# Autodesk Inventor assembly: TrayFeeder
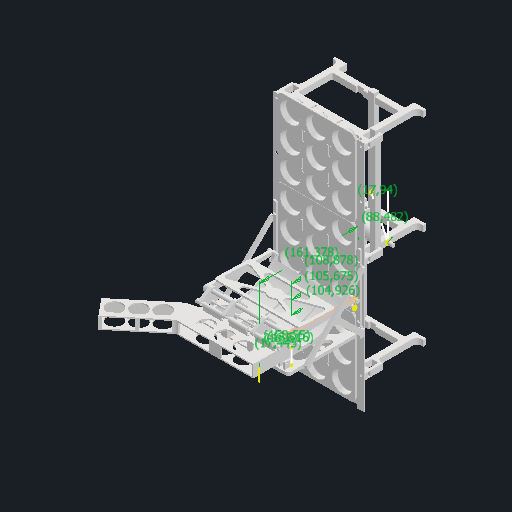
[picture p0: Inventor's stored thumbnail of the model, 512x512]
Saved by Autodesk Inventor 2026 (Build 300175050, 175E)
## iProperties
Created: 2026-05-01
Part Number: TrayFeeder
Document SubType Name: Assembly
Designer: frede
Author: frede
## Documents named in this file (18)
- C:\Users\sniel\OneDrive\SDU\4_Semester\Applied automation\AppliedAutomationProject\feeder\trayFeeder\TrayFeeder.iam
- C:\Users\sniel\OneDrive\SDU\4_Semester\Applied automation\AppliedAutomationProject\feeder\trayFeeder\TrayRail.ipt
- C:\Users\sniel\OneDrive\SDU\4_Semester\Applied automation\AppliedAutomationProject\feeder\trayFeeder\Tray.ipt
- C:\Users\sniel\OneDrive\SDU\4_Semester\Applied automation\AppliedAutomationProject\feeder\trayFeeder\TrayMainLegs.ipt
- C:\Users\sniel\OneDrive\SDU\4_Semester\Applied automation\AppliedAutomationProject\feeder\trayFeeder\Train.ipt
- C:\Users\sniel\OneDrive\SDU\4_Semester\Applied automation\AppliedAutomationProject\feeder\trayFeeder\TrainPullert.ipt
- C:\Users\sniel\OneDrive\SDU\4_Semester\Applied automation\AppliedAutomationProject\feeder\trayFeeder\TrainRail.ipt
- C:\Users\sniel\OneDrive\SDU\4_Semester\Applied automation\AppliedAutomationProject\feeder\trayFeeder\Spacer.ipt
- C:\Users\sniel\OneDrive\SDU\4_Semester\Applied automation\AppliedAutomationProject\feeder\trayFeeder\TrayMainLegs_toPistonWheel.ipt
- C:\Users\sniel\OneDrive\SDU\4_Semester\Applied automation\AppliedAutomationProject\feeder\trayFeeder\Crankshaft.ipt
- C:\Users\sniel\OneDrive\SDU\4_Semester\Applied automation\AppliedAutomationProject\feeder\trayFeeder\ParrallelShaft.ipt
- C:\Users\sniel\OneDrive\SDU\4_Semester\Applied automation\AppliedAutomationProject\feeder\trayFeeder\parrallelShaftPin.ipt
- C:\Users\sniel\OneDrive\SDU\4_Semester\Applied automation\AppliedAutomationProject\feeder\trayFeeder\gaffel.ipt
- C:\Users\sniel\OneDrive\SDU\4_Semester\Applied automation\AppliedAutomationProject\feeder\trayFeeder\ForkTop.ipt
- C:\Users\sniel\OneDrive\SDU\4_Semester\Applied automation\AppliedAutomationProject\feeder\trayFeeder\Ø6x40Shaft.ipt
- C:\Users\sniel\OneDrive\SDU\4_Semester\Applied automation\AppliedAutomationProject\feeder\trayFeeder\LegsStabilizer.ipt
- C:\Users\sniel\OneDrive\SDU\4_Semester\Applied automation\AppliedAutomationProject\feeder\trayFeeder\CoinFeeder.iam
- C:\Users\sniel\OneDrive\SDU\4_Semester\Applied automation\AppliedAutomationProject\feeder\trayFeeder\CoinFeederFoot.ipt
## Components (48 placed, 17 different names)
1. TrayRail:1 — Mate:1, Mate:2, Mate:3, Mate:6, Mate:7, Mate:8, Mate:12, Mate:13, Mate:17, Mate:18, Mate:22, Mate:83, Mate:84, Mate:85, Flush:3, Mate:150, Flush:4
2. Tray:1 — Mate:2, Mate:4, Mate:5, Flush:1, Flush:2
3. Tray:2 — Mate:3, Mate:4, Flush:2
4. Tray:3 — Mate:1, Mate:5, Mate:6, Mate:7, Flush:1
5. TrayMainLegs:1 — Mate:8, Mate:17, Mate:18, Mate:27, Mate:28, Mate:130, Mate:133, Mate:134
6. TrayMainLegs:5 — Mate:12, Mate:13, Mate:22, Mate:30, Mate:124, Mate:125, Mate:126
7. Train:1 — Mate:25, Mate:26, Mate:48, Mate:62, Mate:73, Angle:8, Mate:146
8. TrainPullert:1 — Mate:25, Mate:26
9. TrainRail:1 — Mate:27, Mate:28, Mate:48, Mate:60, Mate:62, Mate:63, Mate:64, Mate:65, Angle:5, Angle:6, Angle:7, Angle:8, Mate:86, Mate:136, Mate:139
10. TrainRail:2 — Mate:30, Mate:56, Mate:57, Mate:58, Mate:59, Mate:66, Mate:67, Mate:68, Mate:69, Angle:1, Angle:2, Angle:3, Angle:4, Mate:87, Mate:88
11. Train:2 — Mate:60, Mate:65, Angle:5, Mate:147
12. TrainPullert:2
13. Train:3 — Mate:35, Mate:64, Angle:6, Mate:136, Mate:137, Mate:138
14. TrainPullert:3 — Mate:35, Mate:137
15. Train:4 — Mate:37, Mate:63, Angle:7, Mate:139, Mate:141, Mate:142
16. TrainPullert:4 — Mate:37, Mate:141
17. Train:5 — Mate:39, Mate:40, Mate:58, Mate:67, Angle:3, Mate:145
18. TrainPullert:5 — Mate:39, Mate:40
19. Train:6 — Mate:59, Mate:66, Angle:4, Mate:148
20. TrainPullert:6
21. Train:7 — Mate:57, Mate:69, Mate:70, Angle:1, Mate:149
22. TrainPullert:7
23. Train:8 — Mate:45, Mate:46, Mate:56, Mate:68, Angle:2, Mate:143, Mate:144
24. TrainPullert:8 — Mate:45, Mate:46
25. Spacer:1 — Mate:70, Mate:100, Mate:148, Mate:149
26. Spacer:2 — Mate:93, Mate:94, Mate:143, Mate:144, Mate:145
27. Spacer:3 — Mate:91, Mate:92, Mate:138, Mate:142
28. Spacer:6 — Mate:73, Mate:97, Mate:140, Mate:146, Mate:147
29. TrayMainLegs_toPistonWheel:1 — Mate:83, Mate:84, Mate:85, Mate:86, Mate:87, Mate:88, Mate:89, Mate:90, Mate:127, Mate:128, Mate:129, Mate:131, Mate:132, Mate:135, Mate:151
30. Crankshaft:1 — Mate:89, Mate:90, Mate:102, Mate:103, Mate:104, Mate:107, Mate:108, Mate:114, Mate:120, Angle:11, Mate:121, Mate:122, Angle:12, Mate:123
31. ParrallelShaft:1 — Mate:93, Mate:94, Mate:98, Angle:10, Mate:99, Mate:105, Mate:111
32. ParrallelShaft:2 — Mate:91, Mate:92, Mate:95, Angle:9, Mate:96, Mate:106, Mate:117, Mate:140
33. parrallelShaftPin:1 — Mate:95, Angle:9, Mate:96, Mate:97
34. parrallelShaftPin:2 — Mate:98, Angle:10, Mate:99, Mate:100
35. gaffel:1 — Mate:103, Mate:104, Mate:105, Mate:112, Mate:113, Mate:115, Mate:116
36. gaffel:2 — Mate:102, Mate:106, Mate:107, Mate:109, Mate:110, Mate:118, Mate:119
37. ForkTop:1 — Mate:108, Mate:109, Mate:110
38. ForkTop:2 — Mate:111, Mate:112, Mate:113
39. ForkTop:3 — Mate:114, Mate:115, Mate:116
40. ForkTop:4 — Mate:117, Mate:118, Mate:119
41. Ø6x40Shaft:1 — Mate:122, Angle:12, Mate:123
42. Ø6x40Shaft:2 — Mate:120, Angle:11, Mate:121
43. LegsStabilizer:1 — Mate:124, Mate:125, Mate:126
44. LegsStabilizer:2 — Mate:127, Mate:128, Mate:129
45. LegsStabilizer:3 — Mate:130, Mate:133, Mate:134
46. LegsStabilizer:4 — Mate:131, Mate:132, Mate:135
47. CoinFeeder:1 [sub-assembly] — Flush:3, Mate:150, Mate:152
48. CoinFeederFoot:1 — Flush:4, Mate:151, Mate:152
## Relationships (131: Mate 115, Angle 12, Flush 4)
- Mate:1: TrayRail:1 ↔ Tray:3
- Mate:2: TrayRail:1 ↔ Tray:1
- Mate:3: TrayRail:1 ↔ Tray:2
- Mate:4: Tray:1 ↔ Tray:2
- Mate:5: Tray:1 ↔ Tray:3
- Mate:6 (19 mm): TrayRail:1 ↔ Tray:3
- Mate:7 (19 mm): TrayRail:1 ↔ Tray:3
- Flush:1: Tray:1 ↔ Tray:3
- Flush:2: Tray:1 ↔ Tray:2
- Mate:8: TrayRail:1 ↔ TrayMainLegs:1
- Mate:12: TrayRail:1 ↔ TrayMainLegs:5
- Mate:13: TrayRail:1 ↔ TrayMainLegs:5
- Mate:17: TrayRail:1 ↔ TrayMainLegs:1
- Mate:18: TrayRail:1 ↔ TrayMainLegs:1
- Mate:22: TrayRail:1 ↔ TrayMainLegs:5
- Mate:25: Train:1 ↔ TrainPullert:1
- Mate:26 (0.1 mm): Train:1 ↔ TrainPullert:1
- Mate:27: TrayMainLegs:1 ↔ TrainRail:1
- Mate:28: TrayMainLegs:1 ↔ TrainRail:1
- Mate:30: TrayMainLegs:5 ↔ TrainRail:2
- [Mate]: Train:2 ↔ TrainPullert:2
- [Mate] (0.1 mm): Train:2 ↔ TrainPullert:2
- Mate:35: Train:3 ↔ TrainPullert:3
- Mate:37: Train:4 ↔ TrainPullert:4
- Mate:39: Train:5 ↔ TrainPullert:5
- Mate:40 (0.1 mm): Train:5 ↔ TrainPullert:5
- [Mate]: Train:6 ↔ TrainPullert:6
- [Mate] (0.1 mm): Train:6 ↔ TrainPullert:6
- [Mate]: Train:7 ↔ TrainPullert:7
- [Mate] (0.1 mm): Train:7 ↔ TrainPullert:7
- Mate:45: Train:8 ↔ TrainPullert:8
- Mate:46 (0.5 mm): Train:8 ↔ TrainPullert:8
- Mate:48 (0.25 mm): Train:1 ↔ TrainRail:1
- Mate:56 (0.25 mm): TrainRail:2 ↔ Train:8
- Mate:57 (0.25 mm): TrainRail:2 ↔ Train:7
- Mate:58 (0.25 mm): TrainRail:2 ↔ Train:5
- Mate:59 (0.25 mm): TrainRail:2 ↔ Train:6
- Mate:60 (0.25 mm): TrainRail:1 ↔ Train:2
- Mate:62 (1 mm): Train:1 ↔ TrainRail:1
- Mate:63 (1 mm): TrainRail:1 ↔ Train:4
- Mate:64 (1 mm): TrainRail:1 ↔ Train:3
- Mate:65 (1 mm): TrainRail:1 ↔ Train:2
- Mate:66 (1 mm): TrainRail:2 ↔ Train:6
- Mate:67 (1 mm): TrainRail:2 ↔ Train:5
- Mate:68 (1 mm): TrainRail:2 ↔ Train:8
- Mate:69 (1 mm): TrainRail:2 ↔ Train:7
- Mate:70: Train:7 ↔ Spacer:1
- Mate:73: Train:1 ↔ Spacer:6
- Angle:1 (0 deg): TrainRail:2 ↔ Train:7
- Angle:2 (0 deg): TrainRail:2 ↔ Train:8
- Angle:3 (0 deg): TrainRail:2 ↔ Train:5
- Angle:4 (0 deg): TrainRail:2 ↔ Train:6
- Angle:5 (0 deg): TrainRail:1 ↔ Train:2
- Angle:6 (0 deg): TrainRail:1 ↔ Train:3
- Angle:7 (0 deg): TrainRail:1 ↔ Train:4
- Angle:8 (0 deg): Train:1 ↔ TrainRail:1
- Mate:83: TrayRail:1 ↔ TrayMainLegs_toPistonWheel:1
- Mate:84: TrayRail:1 ↔ TrayMainLegs_toPistonWheel:1
- Mate:85: TrayRail:1 ↔ TrayMainLegs_toPistonWheel:1
- Mate:86: TrainRail:1 ↔ TrayMainLegs_toPistonWheel:1
- Mate:87: TrainRail:2 ↔ TrayMainLegs_toPistonWheel:1
- Mate:88: TrainRail:2 ↔ TrayMainLegs_toPistonWheel:1
- Mate:89: TrayMainLegs_toPistonWheel:1 ↔ Crankshaft:1
- Mate:90 (0.2 mm): TrayMainLegs_toPistonWheel:1 ↔ Crankshaft:1
- Mate:91: Spacer:3 ↔ ParrallelShaft:2
- Mate:92 (0.125 mm): Spacer:3 ↔ ParrallelShaft:2
- Mate:93: Spacer:2 ↔ ParrallelShaft:1
- Mate:94 (0.125 mm): Spacer:2 ↔ ParrallelShaft:1
- Mate:95: ParrallelShaft:2 ↔ parrallelShaftPin:1
- Angle:9 (180 deg): ParrallelShaft:2 ↔ parrallelShaftPin:1
- Mate:96: ParrallelShaft:2 ↔ parrallelShaftPin:1
- Mate:97: Spacer:6 ↔ parrallelShaftPin:1
- Mate:98: ParrallelShaft:1 ↔ parrallelShaftPin:2
- Angle:10 (180 deg): ParrallelShaft:1 ↔ parrallelShaftPin:2
- Mate:99: ParrallelShaft:1 ↔ parrallelShaftPin:2
- Mate:100: Spacer:1 ↔ parrallelShaftPin:2
- Mate:102 (0.1 mm): Crankshaft:1 ↔ gaffel:2
- Mate:103: Crankshaft:1 ↔ gaffel:1
- Mate:104 (0.1 mm): Crankshaft:1 ↔ gaffel:1
- Mate:105: ParrallelShaft:1 ↔ gaffel:1
- Mate:106: ParrallelShaft:2 ↔ gaffel:2
- Mate:107: Crankshaft:1 ↔ gaffel:2
- Mate:108: Crankshaft:1 ↔ ForkTop:1
- Mate:109: gaffel:2 ↔ ForkTop:1
- Mate:110: gaffel:2 ↔ ForkTop:1
- Mate:111: ParrallelShaft:1 ↔ ForkTop:2
- Mate:112: gaffel:1 ↔ ForkTop:2
- Mate:113: gaffel:1 ↔ ForkTop:2
- Mate:114: Crankshaft:1 ↔ ForkTop:3
- Mate:115: gaffel:1 ↔ ForkTop:3
- Mate:116: gaffel:1 ↔ ForkTop:3
- Mate:117: ParrallelShaft:2 ↔ ForkTop:4
- Mate:118: gaffel:2 ↔ ForkTop:4
- Mate:119: gaffel:2 ↔ ForkTop:4
- Mate:120: Crankshaft:1 ↔ Ø6x40Shaft:2
- Angle:11 (180 deg): Crankshaft:1 ↔ Ø6x40Shaft:2
- Mate:121: Crankshaft:1 ↔ Ø6x40Shaft:2
- Mate:122: Crankshaft:1 ↔ Ø6x40Shaft:1
- Angle:12 (180 deg): Crankshaft:1 ↔ Ø6x40Shaft:1
- Mate:123: Crankshaft:1 ↔ Ø6x40Shaft:1
- Mate:124 (0.05 mm): TrayMainLegs:5 ↔ LegsStabilizer:1
- Mate:125 (0.05 mm): TrayMainLegs:5 ↔ LegsStabilizer:1
- Mate:126: TrayMainLegs:5 ↔ LegsStabilizer:1
- Mate:127: TrayMainLegs_toPistonWheel:1 ↔ LegsStabilizer:2
- Mate:128: TrayMainLegs_toPistonWheel:1 ↔ LegsStabilizer:2
- Mate:129: TrayMainLegs_toPistonWheel:1 ↔ LegsStabilizer:2
- Mate:130: TrayMainLegs:1 ↔ LegsStabilizer:3
- Mate:131: TrayMainLegs_toPistonWheel:1 ↔ LegsStabilizer:4
- Mate:132: TrayMainLegs_toPistonWheel:1 ↔ LegsStabilizer:4
- Mate:133: TrayMainLegs:1 ↔ LegsStabilizer:3
- Mate:134: TrayMainLegs:1 ↔ LegsStabilizer:3
- Mate:135: TrayMainLegs_toPistonWheel:1 ↔ LegsStabilizer:4
- Mate:136 (0.25 mm): TrainRail:1 ↔ Train:3
- Mate:137 (0.5 mm): Train:3 ↔ TrainPullert:3
- Mate:138: Train:3 ↔ Spacer:3
- Mate:139 (0.25 mm): TrainRail:1 ↔ Train:4
- Mate:140: Spacer:6 ↔ ParrallelShaft:2
- Mate:141 (0.5 mm): Train:4 ↔ TrainPullert:4
- Mate:142: Train:4 ↔ Spacer:3
- Mate:143: Train:8 ↔ Spacer:2
- Mate:144: Train:8 ↔ Spacer:2
- Mate:145: Train:5 ↔ Spacer:2
- Mate:146: Train:1 ↔ Spacer:6
- Mate:147: Train:2 ↔ Spacer:6
- Mate:148: Train:6 ↔ Spacer:1
- Mate:149: Train:7 ↔ Spacer:1
- Flush:3 (-166 mm): TrayRail:1 ↔ CoinFeeder:1
- Mate:150 (1.5 mm): TrayRail:1 ↔ CoinFeeder:1
- Flush:4: TrayRail:1 ↔ CoinFeederFoot:1
- Mate:151: TrayMainLegs_toPistonWheel:1 ↔ CoinFeederFoot:1
- Mate:152: CoinFeeder:1 ↔ CoinFeederFoot:1
## Named parameters: d39_d31 = 0 mm, d40_d32 = 0.1 mm, d41_d31 = 0 mm, d43_d31 = 0 mm, d45_d31 = 0 mm, d46_d32 = 0.1 mm, d47_d31 = 0 mm, d48_d32 = 0.1 mm, d49_d31 = 0 mm, d50_d32 = 0.1 mm, d51_d31 = 0 mm, d52_d32 = 0.5 mm
